# Autodesk Inventor assembly: Assembly_Cube_v4_magnet_tshirt
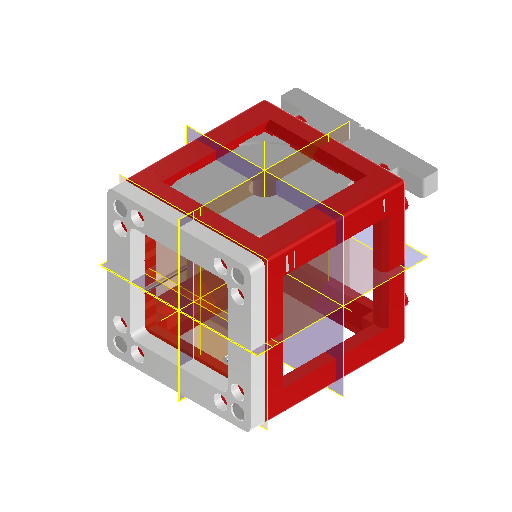
[picture p0: Inventor's stored thumbnail of the model, 512x512]
Saved by Autodesk Inventor 2025.1 (Build 291241020, 241B)
## iProperties
Created: 2024-10-03
Part Number: Assembly_Cube_v4_magnet_tshirt
Document SubType Name: Assembly
Designer: diederichbenedict
Author: diederichbenedict
## Documents named in this file (3)
- C:\Users\diederichbenedict\Dropbox\Dokumente\Promotion\PROJECTS\TechnicalDocs-openUC2-QBox\Production_Files\CAD_Files\INVENTOR\Assembly_Cube_v4_magnet_tshirt.iam
- C:\Users\diederichbenedict\Dropbox\Dokumente\Promotion\PROJECTS\TechnicalDocs-openUC2-QBox\Production_Files\CAD_Files\INVENTOR\Assembly_Cube_v4.iam
- C:\Users\diederichbenedict\Dropbox\Dokumente\Promotion\PROJECTS\TechnicalDocs-openUC2-QBox\Production_Files\CAD_Files\INVENTOR\00_Slider_4_magnet_tshirt.ipt
## Components (2 placed, 2 different names)
1. Assembly_Cube_v4:1 [sub-assembly] — Mate:1, Mate:2, Mate:3
2. 00_Slider_4_magnet_tshirt:1 — Mate:3
## Relationships (3: Mate 3)
- Mate:1: Assembly_Cube_v4:1
- Mate:2: Assembly_Cube_v4:1
- Mate:3: Assembly_Cube_v4:1 ↔ 00_Slider_4_magnet_tshirt:1
